# Autodesk Inventor assembly: FULL SWERVE DRIVE ASSEMBLY!
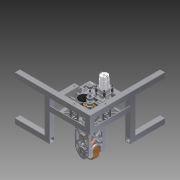
[picture p0: Inventor's stored thumbnail of the model, 180x180]
Saved by Autodesk Inventor 2012 (Build 160160000, 160)
## iProperties
Created: 2012-07-08
Part Number: FULL SWERVE DRIVE ASSEMBLY!
Document SubType Name: Assembly
Designer: Bryce
Author: Bryce
## Documents named in this file (4)
- C:\Users\Bryce\Dropbox\Inventor Design Project Files\Independent Swerves\Inventor 2012\FULL SWERVE DRIVE ASSEMBLY!.iam
- C:\Users\Bryce\Dropbox\Inventor Design Project Files\Independent Swerves\Inventor 2012\Upper gearbox main assembly.iam
- C:\Users\Bryce\Dropbox\Inventor Design Project Files\Independent Swerves\Inventor 2012\Lower box main assembly.iam
- C:\Users\Bryce\Dropbox\Inventor Design Project Files\Independent Swerves\Inventor 2012\frame assembly.iam
## Components (3 placed, 3 different names)
1. Upper gearbox main assembly:1 [sub-assembly] — Mate:1, Flush:1, Mate:2, Mate:3, Mate:4
2. Lower box main assembly:1 [sub-assembly] — Mate:1, Flush:1
3. frame assembly:1 [sub-assembly] — Mate:2, Mate:3, Mate:4
## Relationships (5: Mate 4, Flush 1)
- Mate:1: Upper gearbox main assembly:1 ↔ Lower box main assembly:1
- Flush:1 (-1.5875 mm): Upper gearbox main assembly:1 ↔ Lower box main assembly:1
- Mate:2: Upper gearbox main assembly:1 ↔ frame assembly:1
- Mate:3: Upper gearbox main assembly:1 ↔ frame assembly:1
- Mate:4: Upper gearbox main assembly:1 ↔ frame assembly:1
